# Autodesk Inventor assembly: owl1.1
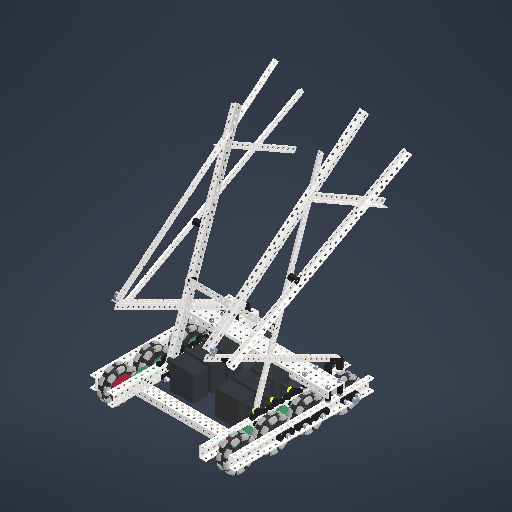
[picture p0: Inventor's stored thumbnail of the model, 512x512]
Saved by Autodesk Inventor 2026 (Build 300175000, 175)
## iProperties
Created: 2025-05-12
Part Number: owl1.1
Document SubType Name: Assembly
Designer: modni
Author: modni
## Documents named in this file (57)
- C:\Vex_cads\owl1.1.iam
- C:\Vex_cads\VEX-CAD-Inventor-1.4.2\Structure\C Channel\Aluminum 1x2x1\Alu C 1x2x1x24.ipt
- C:\Vex_cads\VEX-CAD-Inventor-1.4.2\Motion\Shaft LS\Bearing Flat.ipt
- C:\Vex_cads\VEX-CAD-Inventor-1.4.2\Structure\Hardware\Nut Thin Nylock.ipt
- C:\Vex_cads\VEX-CAD-Inventor-1.4.2\Structure\C Channel\Aluminum 1x3x1\Alu C 1x3x1x25.ipt
- C:\Vex_cads\VEX-CAD-Inventor-1.4.2\Structure\Hardware\Screw Steel - Star\SScrew Star Smooth 1.250.ipt
- C:\Vex_cads\VEX-CAD-Inventor-1.4.2\Structure\Hardware\Screw Steel - Star.ipt
- C:\Vex_cads\VEX-CAD-Inventor-1.4.2\Structure\Hardware\Nut Keps.ipt
- C:\Vex_cads\VEX-CAD-Inventor-1.4.2\Motion\Spacers\Spacer Nylon .375 OD\NSpacer .375 OD x .375.ipt
- C:\Vex_cads\VEX-CAD-Inventor-1.4.2\Motion\Spacers\Spacer Nylon .375 OD.ipt
- C:\Vex_cads\VEX-CAD-Inventor-1.4.2\Structure\C Channel\Aluminum 1x2x1\Alu C 1x2x1x25.ipt
- C:\Vex_cads\VEX-CAD-Inventor-1.4.2\Motion\Shaft LS\Shaft Collar Metal\Shaft Collar Set Screw.ipt
- C:\Vex_cads\VEX-CAD-Inventor-1.4.2\Motion\Spacers\Spacer Nylon .375 OD\NSpacer .375 OD x .250.ipt
- C:\Vex_cads\VEX-CAD-Inventor-1.4.2\Structure\Hardware\Nut Nylock.ipt
- C:\Vex_cads\VEX-CAD-Inventor-1.4.2\Motion\Shaft LS\LS Pillow Bearing Block.ipt
- C:\Vex_cads\VEX-CAD-Inventor-1.4.2\Electronics\V5 Simple Motor.ipt
- C:\Vex_cads\VEX-CAD-Inventor-1.4.2\Motion\Spacers\Washer Teflon\TWasher .375 OD x .04000.ipt
- C:\Vex_cads\VEX-CAD-Inventor-1.4.2\Motion\Spacers\Washer Teflon.ipt
- C:\Vex_cads\VEX-CAD-Inventor-1.4.2\Motion\Spacers\Washer Steel\SWasher .375 OD x .015625.ipt
- C:\Vex_cads\VEX-CAD-Inventor-1.4.2\Motion\Spacers\Washer Steel.ipt
- C:\Vex_cads\VEX-CAD-Inventor-1.4.2\Motion\Wheels\Omni Wheel\2.75 Omni AS, Circle.iam
- C:\Vex_cads\VEX-CAD-Inventor-1.4.2\Motion\Wheels\Omni Wheel.iam
- C:\Vex_cads\VEX-CAD-Inventor-1.4.2\Motion\Gears\HS Gear\HS 36T Gear, Circle.iam
- C:\Vex_cads\VEX-CAD-Inventor-1.4.2\Motion\Gears\HS Gear.iam
- C:\Vex_cads\VEX-CAD-Inventor-1.4.2\Structure\C Channel\Aluminum 1x2x1\Alu C 1x2x1x17.ipt
- C:\Vex_cads\VEX-CAD-Inventor-1.4.2\Motion\Spacers\Spacer Nylon .375 OD\NSpacer .375 OD x .500.ipt
- C:\Vex_cads\VEX-CAD-Inventor-1.4.2\Motion\Gears\LS 36T Gear.ipt
- C:\Vex_cads\VEX-CAD-Inventor-1.4.2\Motion\Wheels\Omni Wheel\2.75 Omni AS, Square.iam
- C:\Vex_cads\VEX-CAD-Inventor-1.4.2\Structure\C Channel\Aluminum 1x2x1\Alu C 1x2x1x24_MIR.ipt
- C:\Vex_cads\VEX-CAD-Inventor-1.4.2\Motion\Shaft LS\Bearing Flat_MIR.ipt
- C:\Vex_cads\VEX-CAD-Inventor-1.4.2\Structure\Hardware\Nut Thin Nylock_MIR.ipt
- C:\Vex_cads\VEX-CAD-Inventor-1.4.2\Structure\Hardware\Nut Keps_MIR.ipt
- C:\Vex_cads\VEX-CAD-Inventor-1.4.2\Structure\C Channel\Aluminum 1x2x1\Alu C 1x2x1x25_MIR.ipt
- C:\Vex_cads\VEX-CAD-Inventor-1.4.2\Motion\Shaft LS\Shaft Collar Metal\Shaft Collar Set Screw_MIR.ipt
- C:\Vex_cads\VEX-CAD-Inventor-1.4.2\Structure\Hardware\Nut Nylock_MIR.ipt
- C:\Vex_cads\VEX-CAD-Inventor-1.4.2\Motion\Shaft LS\LS Pillow Bearing Block_MIR.ipt
- C:\Vex_cads\VEX-CAD-Inventor-1.4.2\Electronics\V5 Simple Motor_MIR.ipt
- C:\Vex_cads\VEX-CAD-Inventor-1.4.2\Motion\Wheels\Omni Wheel\2.75 Omni AS, Circle_MIR.iam
- C:\Vex_cads\VEX-CAD-Inventor-1.4.2\Motion\Gears\HS Gear\HS 36T Gear, Circle_MIR.iam
- C:\Vex_cads\VEX-CAD-Inventor-1.4.2\Motion\Gears\LS 36T Gear_MIR.ipt
- C:\Vex_cads\VEX-CAD-Inventor-1.4.2\Motion\Wheels\Omni Wheel\2.75 Omni AS, Square_MIR.iam
- C:\Vex_cads\VEX-CAD-Inventor-1.4.2\Motion\Spacers\Spacer Nylon .500 OD\NSpacer Black .500 OD x .500.ipt
- C:\Vex_cads\VEX-CAD-Inventor-1.4.2\Motion\Spacers\Spacer Nylon .500 OD.ipt
- C:\Vex_cads\VEX-CAD-Inventor-1.4.2\Motion\Spacers\Spacer Nylon .500 OD\NSpacer Black .500 OD x .125.ipt
- C:\Vex_cads\VEX-CAD-Inventor-1.4.2\Structure\Angle\Aluminum 1x1\Alu Angle 1x1x25.ipt
- C:\Vex_cads\VEX-CAD-Inventor-1.4.2\Structure\Angle\Aluminum 1x1\Alu Angle 1x1x35.ipt
- C:\Vex_cads\VEX-CAD-Inventor-1.4.2\Motion\Spacers\Spacer Nylon .375 OD\NSpacer .375 OD x .125.ipt
- C:\Vex_cads\VEX-CAD-Inventor-1.4.2\Motion\Spacers\Spacer Nylon .500 OD\NSpacer Black .500 OD x .375.ipt
- C:\Vex_cads\VEX-CAD-Inventor-1.4.2\Motion\Spacers\Spacer Nylon .500 OD\NSpacer Black .500 OD x .250.ipt
- C:\Vex_cads\VEX-CAD-Inventor-1.4.2\Motion\Shaft LS\Shaft Collar Metal\Shaft Collar No Screw.ipt
- C:\Vex_cads\VEX-CAD-Inventor-1.4.2\Structure\Angle\Aluminum 1x1\Alu Angle 1x1x15.ipt
- C:\Vex_cads\VEX-CAD-Inventor-1.4.2\Motion\Shaft LS\LS Pillow Bearing Block_MIR1.ipt
- C:\Vex_cads\VEX-CAD-Inventor-1.4.2\Structure\Angle\Aluminum 1x1\Alu Angle 1x1x25_MIR.ipt
- C:\Vex_cads\VEX-CAD-Inventor-1.4.2\Structure\Angle\Aluminum 1x1\Alu Angle 1x1x35_MIR.ipt
- C:\Vex_cads\VEX-CAD-Inventor-1.4.2\Motion\Shaft LS\Shaft Collar Metal\Shaft Collar No Screw_MIR.ipt
- C:\Vex_cads\VEX-CAD-Inventor-1.4.2\Structure\Hardware\Nut Keps_MIR1.ipt
- C:\Vex_cads\VEX-CAD-Inventor-1.4.2\Structure\Angle\Aluminum 1x1\Alu Angle 1x1x15_MIR.ipt
## Components (193 placed, 49 different names)
1. Alu C 1x2x1x24:1 — Mate:1, Mate:2, Mate:3, Mate:4, Insert:2, Insert:3, Insert:4, Insert:5, Symmetry:1
2. Bearing Flat:1 — Mate:1, Mate:6
3. Bearing Flat:2 — Mate:2, Mate:5
4. Bearing Flat:3 — Mate:3, Mate:7
5. Bearing Flat:4 — Mate:4, Mate:8, Insert:1, Insert:25
6. Nut Thin Nylock:1 — Mate:6
7. Nut Thin Nylock:2 — Mate:5
8. Nut Thin Nylock:3 — Mate:7
9. Nut Thin Nylock:4 — Insert:1
10. Nut Thin Nylock:5 — Mate:8
11. Alu C 1x3x1x25:1 — Insert:10, Insert:15, Insert:16, Insert:33, Insert:34, Insert:35, Insert:36
12. SScrew Star Smooth 1.250:1 — Insert:3
13. SScrew Star Smooth 1.250:2 — Insert:2
14. Nut Keps:1 — Insert:5, Insert:8
15. Nut Keps:2 — Insert:4, Insert:6
16. NSpacer .375 OD x .375:1 — Insert:6, Insert:7
17. NSpacer .375 OD x .375:2 — Insert:7
18. NSpacer .375 OD x .375:3 — Insert:9, Insert:10
19. NSpacer .375 OD x .375:4 — Insert:8, Insert:9
20. Alu C 1x2x1x25:1 — Insert:17, Insert:18, Insert:19, Insert:20, Insert:21, Insert:22, Insert:23, Insert:37, Insert:38, Insert:39, Insert:40, Insert:41, Insert:42, Insert:50, Insert:55, Insert:56, Insert:70, Insert:71, Insert:72, Insert:76, Insert:77, Insert:141, Insert:143
21. SScrew Star Smooth 1.250:3 — Insert:19
22. SScrew Star Smooth 1.250:4 — Insert:18
23. Nut Keps:3 — Insert:17
24. Nut Keps:4
25. NSpacer .375 OD x .375:5
26. NSpacer .375 OD x .375:6 — Insert:15
27. NSpacer .375 OD x .375:7 — Insert:16
28. NSpacer .375 OD x .375:8
29. Bearing Flat:5 — Insert:23, Insert:24
30. Bearing Flat:6 — Insert:22, Insert:31, Insert:32
31. Bearing Flat:7 — Insert:21, Insert:29, Insert:30
32. Bearing Flat:8 — Insert:20, Insert:27, Insert:28
33. Shaft Collar Set Screw:1 — Insert:24
34. Shaft Collar Set Screw:2 — Insert:26
35. NSpacer .375 OD x .250:9 — Insert:25, Insert:26
36. Nut Nylock:1 — Insert:32
37. Nut Nylock:2 — Insert:31
38. Nut Nylock:3 — Insert:30
39. Nut Nylock:4 — Insert:29
40. Nut Nylock:5 — Insert:27
41. Nut Nylock:6 — Insert:28
42. Nut Thin Nylock:6 — Insert:33
43. Nut Thin Nylock:7 — Insert:34
44. Nut Thin Nylock:8 — Insert:35
45. Nut Thin Nylock:9 — Insert:36
46. LS Pillow Bearing Block:1 — Insert:37, Insert:147
47. LS Pillow Bearing Block:2 — Insert:38
48. LS Pillow Bearing Block:3 — Insert:39
49. V5 Simple Motor:1 — Insert:40
50. V5 Simple Motor:2 — Insert:41
51. V5 Simple Motor:3 — Insert:42
52. NSpacer .375 OD x .250:10 — Insert:49
53. TWasher .375 OD x .04000:1 — Insert:43, Insert:54
54. SWasher .375 OD x .015625:1 — Insert:43, Insert:51
55. 2.75 Omni AS, Circle:1 [sub-assembly] — Insert:49, Insert:52
56. Nut Keps:5 — Insert:50, Insert:53
57. HS 36T Gear, Circle:1 [sub-assembly] — Insert:51, Insert:52
58. NSpacer .375 OD x .375:11 — Insert:53, Insert:54
59. Alu C 1x2x1x17:1 — Insert:55
60. NSpacer .375 OD x .250:14 — Insert:60, Insert:61
61. NSpacer .375 OD x .500:12 — Insert:56, Insert:57
62. LS 36T Gear:1 — Insert:57, Insert:60
63. 2.75 Omni AS, Square:3 [sub-assembly] — Insert:59, Insert:61
64. NSpacer .375 OD x .375:13 — Insert:59
65. NSpacer .375 OD x .500:15 — Insert:70
66. LS 36T Gear:2
67. 2.75 Omni AS, Square:4 [sub-assembly]
68. NSpacer .375 OD x .375:16
69. NSpacer .375 OD x .250:17
70. NSpacer .375 OD x .500:18 — Insert:71
71. LS 36T Gear:3
72. 2.75 Omni AS, Square:5 [sub-assembly]
73. NSpacer .375 OD x .375:19
74. NSpacer .375 OD x .250:20
75. NSpacer .375 OD x .500:21 — Insert:72, Insert:73
76. LS 36T Gear:4 — Insert:73
77. NSpacer .375 OD x .500:22 — Insert:77
78. LS 36T Gear:5
79. NSpacer .375 OD x .500:23 — Insert:76
80. LS 36T Gear:6
81. Alu C 1x2x1x24_MIR:1 — Mate:9, Mate:10, Mate:11, Mate:12, Insert:79, Insert:80, Insert:81, Insert:82, Symmetry:1
82. Bearing Flat_MIR:1 — Mate:9, Mate:13
83. Bearing Flat_MIR:2 — Mate:10, Mate:14
84. Bearing Flat_MIR:3 — Mate:11, Mate:15
85. Bearing Flat_MIR:4 — Mate:12, Insert:78, Mate:16, Insert:100
86. Nut Thin Nylock_MIR:1 — Mate:13
87. Nut Thin Nylock_MIR:2 — Mate:14
88. Nut Thin Nylock_MIR:3 — Mate:15
89. Nut Thin Nylock_MIR:4 — Insert:78
90. Nut Thin Nylock_MIR:5 — Mate:16
91. SScrew Star Smooth 1.250:5 — Insert:79
92. SScrew Star Smooth 1.250:6 — Insert:80
93. Nut Keps_MIR:1 — Insert:81, Insert:86
94. Nut Keps_MIR:2 — Insert:82, Insert:83
95. NSpacer .375 OD x .375:24 — Insert:83, Insert:84
96. NSpacer .375 OD x .375:25 — Insert:84
97. NSpacer .375 OD x .375:26 — Insert:85
98. NSpacer .375 OD x .375:27 — Insert:85, Insert:86
99. Alu C 1x2x1x25_MIR:1 — Insert:87, Insert:88, Insert:89, Insert:94, Insert:95, Insert:96, Insert:97, Insert:107, Insert:108, Insert:109, Insert:110, Insert:111, Insert:112, Insert:115, Insert:120, Insert:125, Insert:130, Insert:135, Insert:137, Insert:139
100. SScrew Star Smooth 1.250:7 — Insert:87
101. SScrew Star Smooth 1.250:8 — Insert:88
102. Nut Keps_MIR:3 — Insert:89, Insert:93
103. Nut Keps_MIR:4 — Insert:90
104. NSpacer .375 OD x .375:28 — Insert:90, Insert:91
105. NSpacer .375 OD x .375:29 — Insert:91
106. NSpacer .375 OD x .375:30 — Insert:92
107. NSpacer .375 OD x .375:31 — Insert:92, Insert:93
108. Bearing Flat_MIR:5 — Insert:94, Insert:98
109. Bearing Flat_MIR:6 — Insert:95, Insert:101, Insert:102
110. Bearing Flat_MIR:7 — Insert:96, Insert:103, Insert:104
111. Bearing Flat_MIR:8 — Insert:97, Insert:105, Insert:106
112. Shaft Collar Set Screw_MIR:1 — Insert:98
113. Shaft Collar Set Screw_MIR:2 — Insert:99
114. NSpacer .375 OD x .250:32 — Insert:99, Insert:100
115. Nut Nylock_MIR:1 — Insert:101
116. Nut Nylock_MIR:2 — Insert:102
117. Nut Nylock_MIR:3 — Insert:103
118. Nut Nylock_MIR:4 — Insert:104
119. Nut Nylock_MIR:5 — Insert:105
120. Nut Nylock_MIR:6 — Insert:106
121. Nut Thin Nylock_MIR:6
122. Nut Thin Nylock_MIR:7
123. Nut Thin Nylock_MIR:8
124. Nut Thin Nylock_MIR:9
125. LS Pillow Bearing Block_MIR:1 — Insert:107
126. LS Pillow Bearing Block_MIR:2 — Insert:108
127. LS Pillow Bearing Block_MIR:3 — Insert:109
128. V5 Simple Motor_MIR:1 — Insert:110
129. V5 Simple Motor_MIR:2 — Insert:111
130. V5 Simple Motor_MIR:3 — Insert:112
131. NSpacer .375 OD x .250:33 — Insert:114
132. TWasher .375 OD x .04000:2 — Insert:113, Insert:118
133. SWasher .375 OD x .015625:2 — Insert:113, Insert:117
134. 2.75 Omni AS, Circle_MIR:1 [sub-assembly] — Insert:114, Insert:116
135. Nut Keps_MIR:5 — Insert:115, Insert:119
136. HS 36T Gear, Circle_MIR:1 [sub-assembly] — Insert:116, Insert:117
137. NSpacer .375 OD x .375:34 — Insert:118, Insert:119
138. NSpacer .375 OD x .250:35 — Insert:123, Insert:124
139. NSpacer .375 OD x .500:36 — Insert:120, Insert:121
140. LS 36T Gear_MIR:1 — Insert:121, Insert:124
141. 2.75 Omni AS, Square_MIR:1 [sub-assembly] — Insert:122, Insert:123
142. NSpacer .375 OD x .375:37 — Insert:122
143. NSpacer .375 OD x .500:38 — Insert:125, Insert:126
144. LS 36T Gear_MIR:2 — Insert:126, Insert:129
145. 2.75 Omni AS, Square_MIR:2 [sub-assembly] — Insert:127, Insert:128
146. NSpacer .375 OD x .375:39 — Insert:127
147. NSpacer .375 OD x .250:40 — Insert:128, Insert:129
148. NSpacer .375 OD x .500:41 — Insert:130, Insert:131
149. LS 36T Gear_MIR:3 — Insert:131, Insert:134
150. 2.75 Omni AS, Square_MIR:3 [sub-assembly] — Insert:132, Insert:133
151. NSpacer .375 OD x .375:42 — Insert:132
152. NSpacer .375 OD x .250:43 — Insert:133, Insert:134
153. NSpacer .375 OD x .500:44 — Insert:135, Insert:136
154. LS 36T Gear_MIR:4 — Insert:136
155. NSpacer .375 OD x .500:45 — Insert:137, Insert:138
156. LS 36T Gear_MIR:5 — Insert:138
157. NSpacer .375 OD x .500:46 — Insert:139, Insert:140
158. LS 36T Gear_MIR:6 — Insert:140
159. NSpacer Black .500 OD x .500:1 — Insert:141, Insert:142
160. NSpacer Black .500 OD x .500:2 — Insert:143, Insert:144
161. NSpacer Black .500 OD x .125:3 — Insert:142, Insert:145
162. NSpacer Black .500 OD x .125:4 — Insert:144
163. LS Pillow Bearing Block:4 — Insert:145, Insert:146
164. Alu Angle 1x1x25:1 — Insert:146, Insert:149, Insert:150, Insert:154
165. Alu Angle 1x1x35:1 — Insert:148, Insert:149, Insert:152, Insert:157, Insert:172
166. NSpacer .375 OD x .125:47 — Insert:147, Insert:148
167. Alu Angle 1x1x35:2 — Insert:151
168. NSpacer .375 OD x .500:48 — Insert:150, Insert:151
169. NSpacer Black .500 OD x .375:6 — Insert:153
170. NSpacer Black .500 OD x .250:7 — Insert:152, Insert:153
171. Alu Angle 1x1x35:3 — Insert:156
172. Shaft Collar No Screw:1 — Insert:155, Insert:156
173. Nut Keps:6 — Insert:154, Insert:155
174. Alu Angle 1x1x15:1 — Insert:157
175. NSpacer Black .500 OD x .500:8 — Insert:158
176. NSpacer Black .500 OD x .500:9 — Insert:159
177. NSpacer Black .500 OD x .125:10 — Insert:158, Insert:160
178. NSpacer Black .500 OD x .125:11 — Insert:159
179. LS Pillow Bearing Block_MIR1:1 — Insert:160, Insert:161
180. Alu Angle 1x1x25_MIR:1 — Insert:161, Insert:162, Insert:165, Insert:170
181. Alu Angle 1x1x35_MIR:1 — Insert:162, Insert:163, Insert:167, Insert:171, Insert:173
182. NSpacer .375 OD x .125:49 — Insert:163
183. Alu Angle 1x1x35_MIR:2 — Insert:164
184. NSpacer .375 OD x .500:50 — Insert:164, Insert:165
185. NSpacer Black .500 OD x .375:12 — Insert:166
186. NSpacer Black .500 OD x .250:13 — Insert:166, Insert:167
187. Alu Angle 1x1x35_MIR:3 — Insert:168
188. Shaft Collar No Screw_MIR:1 — Insert:168, Insert:169
189. Nut Keps_MIR1:1 — Insert:169, Insert:170
190. Alu Angle 1x1x15_MIR:1 — Insert:171
191. NSpacer .375 OD x .500:51 — Insert:172, Insert:174
192. NSpacer .375 OD x .500:52 — Insert:173, Insert:175
193. Alu Angle 1x1x15:2 — Insert:174, Insert:175
## Relationships (186: Insert 169, Mate 16, Symmetry 1)
- Mate:1: Alu C 1x2x1x24:1 ↔ Bearing Flat:1
- Mate:2: Alu C 1x2x1x24:1 ↔ Bearing Flat:2
- Mate:3: Alu C 1x2x1x24:1 ↔ Bearing Flat:3
- Mate:4: Alu C 1x2x1x24:1 ↔ Bearing Flat:4
- Mate:5: Bearing Flat:2 ↔ Nut Thin Nylock:2
- Mate:6: Bearing Flat:1 ↔ Nut Thin Nylock:1
- Mate:7: Bearing Flat:3 ↔ Nut Thin Nylock:3
- Mate:8: Bearing Flat:4 ↔ Nut Thin Nylock:5
- Insert:1: Bearing Flat:4 ↔ Nut Thin Nylock:4
- Insert:2: Alu C 1x2x1x24:1 ↔ SScrew Star Smooth 1.250:2
- Insert:3: Alu C 1x2x1x24:1 ↔ SScrew Star Smooth 1.250:1
- Insert:4: Alu C 1x2x1x24:1 ↔ Nut Keps:2
- Insert:5: Alu C 1x2x1x24:1 ↔ Nut Keps:1
- Insert:6: Nut Keps:2 ↔ NSpacer .375 OD x .375:1
- Insert:7: NSpacer .375 OD x .375:1 ↔ NSpacer .375 OD x .375:2
- Insert:8: Nut Keps:1 ↔ NSpacer .375 OD x .375:4
- Insert:9: NSpacer .375 OD x .375:3 ↔ NSpacer .375 OD x .375:4
- Insert:10: Alu C 1x3x1x25:1 ↔ NSpacer .375 OD x .375:3
- [Insert]: Nut Keps:4 ↔ NSpacer .375 OD x .375:5
- [Insert]: NSpacer .375 OD x .375:5 ↔ NSpacer .375 OD x .375:6
- [Insert]: Nut Keps:3 ↔ NSpacer .375 OD x .375:8
- [Insert]: NSpacer .375 OD x .375:7 ↔ NSpacer .375 OD x .375:8
- Insert:15: Alu C 1x3x1x25:1 ↔ NSpacer .375 OD x .375:6
- Insert:16: Alu C 1x3x1x25:1 ↔ NSpacer .375 OD x .375:7
- Insert:17: Alu C 1x2x1x25:1 ↔ Nut Keps:3
- Insert:18: Alu C 1x2x1x25:1 ↔ SScrew Star Smooth 1.250:4
- Insert:19: Alu C 1x2x1x25:1 ↔ SScrew Star Smooth 1.250:3
- Insert:20: Alu C 1x2x1x25:1 ↔ Bearing Flat:8
- Insert:21: Alu C 1x2x1x25:1 ↔ Bearing Flat:7
- Insert:22: Alu C 1x2x1x25:1 ↔ Bearing Flat:6
- Insert:23: Alu C 1x2x1x25:1 ↔ Bearing Flat:5
- Insert:24: Bearing Flat:5 ↔ Shaft Collar Set Screw:1
- Insert:25: Bearing Flat:4 ↔ NSpacer .375 OD x .250:9
- Insert:26: Shaft Collar Set Screw:2 ↔ NSpacer .375 OD x .250:9
- Insert:27: Bearing Flat:8 ↔ Nut Nylock:5
- Insert:28: Bearing Flat:8 ↔ Nut Nylock:6
- Insert:29: Bearing Flat:7 ↔ Nut Nylock:4
- Insert:30: Bearing Flat:7 ↔ Nut Nylock:3
- Insert:31: Bearing Flat:6 ↔ Nut Nylock:2
- Insert:32: Bearing Flat:6 ↔ Nut Nylock:1
- Insert:33: Alu C 1x3x1x25:1 ↔ Nut Thin Nylock:6
- Insert:34: Alu C 1x3x1x25:1 ↔ Nut Thin Nylock:7
- Insert:35: Alu C 1x3x1x25:1 ↔ Nut Thin Nylock:8
- Insert:36: Alu C 1x3x1x25:1 ↔ Nut Thin Nylock:9
- Insert:37: Alu C 1x2x1x25:1 ↔ LS Pillow Bearing Block:1
- Insert:38: Alu C 1x2x1x25:1 ↔ LS Pillow Bearing Block:2
- Insert:39: Alu C 1x2x1x25:1 ↔ LS Pillow Bearing Block:3
- Insert:40: Alu C 1x2x1x25:1 ↔ V5 Simple Motor:1
- Insert:41: Alu C 1x2x1x25:1 ↔ V5 Simple Motor:2
- Insert:42: Alu C 1x2x1x25:1 ↔ V5 Simple Motor:3
- Insert:43: TWasher .375 OD x .04000:1 ↔ SWasher .375 OD x .015625:1
- Insert:49: NSpacer .375 OD x .250:10 ↔ 2.75 Omni AS, Circle:1
- Insert:50: Alu C 1x2x1x25:1 ↔ Nut Keps:5
- Insert:51: SWasher .375 OD x .015625:1 ↔ HS 36T Gear, Circle:1
- Insert:52: 2.75 Omni AS, Circle:1 ↔ HS 36T Gear, Circle:1
- Insert:53: Nut Keps:5 ↔ NSpacer .375 OD x .375:11
- Insert:54: TWasher .375 OD x .04000:1 ↔ NSpacer .375 OD x .375:11
- Insert:55: Alu C 1x2x1x25:1 ↔ Alu C 1x2x1x17:1
- Insert:56: Alu C 1x2x1x25:1 ↔ NSpacer .375 OD x .500:12
- Insert:57: NSpacer .375 OD x .500:12 ↔ LS 36T Gear:1
- Insert:59: 2.75 Omni AS, Square:3 ↔ NSpacer .375 OD x .375:13
- Insert:60: NSpacer .375 OD x .250:14 ↔ LS 36T Gear:1
- Insert:61: NSpacer .375 OD x .250:14 ↔ 2.75 Omni AS, Square:3
- [Insert]: NSpacer .375 OD x .500:15 ↔ LS 36T Gear:2
- [Insert]: 2.75 Omni AS, Square:4 ↔ NSpacer .375 OD x .375:16
- [Insert]: LS 36T Gear:2 ↔ NSpacer .375 OD x .250:17
- [Insert]: 2.75 Omni AS, Square:4 ↔ NSpacer .375 OD x .250:17
- [Insert]: NSpacer .375 OD x .500:18 ↔ LS 36T Gear:3
- [Insert]: 2.75 Omni AS, Square:5 ↔ NSpacer .375 OD x .375:19
- [Insert]: LS 36T Gear:3 ↔ NSpacer .375 OD x .250:20
- [Insert]: 2.75 Omni AS, Square:5 ↔ NSpacer .375 OD x .250:20
- Insert:70: Alu C 1x2x1x25:1 ↔ NSpacer .375 OD x .500:15
- Insert:71: Alu C 1x2x1x25:1 ↔ NSpacer .375 OD x .500:18
- Insert:72: Alu C 1x2x1x25:1 ↔ NSpacer .375 OD x .500:21
- Insert:73: NSpacer .375 OD x .500:21 ↔ LS 36T Gear:4
- [Insert]: NSpacer .375 OD x .500:22 ↔ LS 36T Gear:5
- [Insert]: NSpacer .375 OD x .500:23 ↔ LS 36T Gear:6
- Insert:76: Alu C 1x2x1x25:1 ↔ NSpacer .375 OD x .500:23
- Insert:77: Alu C 1x2x1x25:1 ↔ NSpacer .375 OD x .500:22
- Mate:9: Alu C 1x2x1x24_MIR:1 ↔ Bearing Flat_MIR:1
- Mate:10: Alu C 1x2x1x24_MIR:1 ↔ Bearing Flat_MIR:2
- Mate:11: Alu C 1x2x1x24_MIR:1 ↔ Bearing Flat_MIR:3
- Mate:12: Alu C 1x2x1x24_MIR:1 ↔ Bearing Flat_MIR:4
- Mate:13: Bearing Flat_MIR:1 ↔ Nut Thin Nylock_MIR:1
- Mate:14: Bearing Flat_MIR:2 ↔ Nut Thin Nylock_MIR:2
- Mate:15: Bearing Flat_MIR:3 ↔ Nut Thin Nylock_MIR:3
- Insert:78: Bearing Flat_MIR:4 ↔ Nut Thin Nylock_MIR:4
- Mate:16: Bearing Flat_MIR:4 ↔ Nut Thin Nylock_MIR:5
- Insert:79: Alu C 1x2x1x24_MIR:1 ↔ SScrew Star Smooth 1.250:5
- Insert:80: Alu C 1x2x1x24_MIR:1 ↔ SScrew Star Smooth 1.250:6
- Insert:81: Alu C 1x2x1x24_MIR:1 ↔ Nut Keps_MIR:1
- Insert:82: Alu C 1x2x1x24_MIR:1 ↔ Nut Keps_MIR:2
- Insert:83: Nut Keps_MIR:2 ↔ NSpacer .375 OD x .375:24
- Insert:84: NSpacer .375 OD x .375:24 ↔ NSpacer .375 OD x .375:25
- Insert:85: NSpacer .375 OD x .375:26 ↔ NSpacer .375 OD x .375:27
- Insert:86: Nut Keps_MIR:1 ↔ NSpacer .375 OD x .375:27
- Insert:87: Alu C 1x2x1x25_MIR:1 ↔ SScrew Star Smooth 1.250:7
- Insert:88: Alu C 1x2x1x25_MIR:1 ↔ SScrew Star Smooth 1.250:8
- Insert:89: Alu C 1x2x1x25_MIR:1 ↔ Nut Keps_MIR:3
- Insert:90: Nut Keps_MIR:4 ↔ NSpacer .375 OD x .375:28
- Insert:91: NSpacer .375 OD x .375:28 ↔ NSpacer .375 OD x .375:29
- Insert:92: NSpacer .375 OD x .375:30 ↔ NSpacer .375 OD x .375:31
- Insert:93: Nut Keps_MIR:3 ↔ NSpacer .375 OD x .375:31
- Insert:94: Alu C 1x2x1x25_MIR:1 ↔ Bearing Flat_MIR:5
- Insert:95: Alu C 1x2x1x25_MIR:1 ↔ Bearing Flat_MIR:6
- Insert:96: Alu C 1x2x1x25_MIR:1 ↔ Bearing Flat_MIR:7
- Insert:97: Alu C 1x2x1x25_MIR:1 ↔ Bearing Flat_MIR:8
- Insert:98: Bearing Flat_MIR:5 ↔ Shaft Collar Set Screw_MIR:1
- Insert:99: Shaft Collar Set Screw_MIR:2 ↔ NSpacer .375 OD x .250:32
- Insert:100: Bearing Flat_MIR:4 ↔ NSpacer .375 OD x .250:32
- Insert:101: Bearing Flat_MIR:6 ↔ Nut Nylock_MIR:1
- Insert:102: Bearing Flat_MIR:6 ↔ Nut Nylock_MIR:2
- Insert:103: Bearing Flat_MIR:7 ↔ Nut Nylock_MIR:3
- Insert:104: Bearing Flat_MIR:7 ↔ Nut Nylock_MIR:4
- Insert:105: Bearing Flat_MIR:8 ↔ Nut Nylock_MIR:5
- Insert:106: Bearing Flat_MIR:8 ↔ Nut Nylock_MIR:6
- Insert:107: Alu C 1x2x1x25_MIR:1 ↔ LS Pillow Bearing Block_MIR:1
- Insert:108: Alu C 1x2x1x25_MIR:1 ↔ LS Pillow Bearing Block_MIR:2
- Insert:109: Alu C 1x2x1x25_MIR:1 ↔ LS Pillow Bearing Block_MIR:3
- Insert:110: Alu C 1x2x1x25_MIR:1 ↔ V5 Simple Motor_MIR:1
- Insert:111: Alu C 1x2x1x25_MIR:1 ↔ V5 Simple Motor_MIR:2
- Insert:112: Alu C 1x2x1x25_MIR:1 ↔ V5 Simple Motor_MIR:3
- Insert:113: TWasher .375 OD x .04000:2 ↔ SWasher .375 OD x .015625:2
- Insert:114: NSpacer .375 OD x .250:33 ↔ 2.75 Omni AS, Circle_MIR:1
- Insert:115: Alu C 1x2x1x25_MIR:1 ↔ Nut Keps_MIR:5
- Insert:116: 2.75 Omni AS, Circle_MIR:1 ↔ HS 36T Gear, Circle_MIR:1
- Insert:117: SWasher .375 OD x .015625:2 ↔ HS 36T Gear, Circle_MIR:1
- Insert:118: TWasher .375 OD x .04000:2 ↔ NSpacer .375 OD x .375:34
- Insert:119: Nut Keps_MIR:5 ↔ NSpacer .375 OD x .375:34
- Insert:120: Alu C 1x2x1x25_MIR:1 ↔ NSpacer .375 OD x .500:36
- Insert:121: NSpacer .375 OD x .500:36 ↔ LS 36T Gear_MIR:1
- Insert:122: 2.75 Omni AS, Square_MIR:1 ↔ NSpacer .375 OD x .375:37
- Insert:123: NSpacer .375 OD x .250:35 ↔ 2.75 Omni AS, Square_MIR:1
- Insert:124: NSpacer .375 OD x .250:35 ↔ LS 36T Gear_MIR:1
- Insert:125: Alu C 1x2x1x25_MIR:1 ↔ NSpacer .375 OD x .500:38
- Insert:126: NSpacer .375 OD x .500:38 ↔ LS 36T Gear_MIR:2
- Insert:127: 2.75 Omni AS, Square_MIR:2 ↔ NSpacer .375 OD x .375:39
- Insert:128: 2.75 Omni AS, Square_MIR:2 ↔ NSpacer .375 OD x .250:40
- Insert:129: LS 36T Gear_MIR:2 ↔ NSpacer .375 OD x .250:40
- Insert:130: Alu C 1x2x1x25_MIR:1 ↔ NSpacer .375 OD x .500:41
- Insert:131: NSpacer .375 OD x .500:41 ↔ LS 36T Gear_MIR:3
- Insert:132: 2.75 Omni AS, Square_MIR:3 ↔ NSpacer .375 OD x .375:42
- Insert:133: 2.75 Omni AS, Square_MIR:3 ↔ NSpacer .375 OD x .250:43
- Insert:134: LS 36T Gear_MIR:3 ↔ NSpacer .375 OD x .250:43
- Insert:135: Alu C 1x2x1x25_MIR:1 ↔ NSpacer .375 OD x .500:44
- Insert:136: NSpacer .375 OD x .500:44 ↔ LS 36T Gear_MIR:4
- Insert:137: Alu C 1x2x1x25_MIR:1 ↔ NSpacer .375 OD x .500:45
- Insert:138: NSpacer .375 OD x .500:45 ↔ LS 36T Gear_MIR:5
- Insert:139: Alu C 1x2x1x25_MIR:1 ↔ NSpacer .375 OD x .500:46
- Insert:140: NSpacer .375 OD x .500:46 ↔ LS 36T Gear_MIR:6
- Insert:141: Alu C 1x2x1x25:1 ↔ NSpacer Black .500 OD x .500:1
- Insert:142: NSpacer Black .500 OD x .500:1 ↔ NSpacer Black .500 OD x .125:3
- Insert:143: Alu C 1x2x1x25:1 ↔ NSpacer Black .500 OD x .500:2
- Insert:144: NSpacer Black .500 OD x .500:2 ↔ NSpacer Black .500 OD x .125:4
- Insert:145: NSpacer Black .500 OD x .125:3 ↔ LS Pillow Bearing Block:4
- Insert:146: LS Pillow Bearing Block:4 ↔ Alu Angle 1x1x25:1
- Insert:147: LS Pillow Bearing Block:1 ↔ NSpacer .375 OD x .125:47
- Insert:148: Alu Angle 1x1x35:1 ↔ NSpacer .375 OD x .125:47
- Insert:149: Alu Angle 1x1x25:1 ↔ Alu Angle 1x1x35:1
- Insert:150: Alu Angle 1x1x25:1 ↔ NSpacer .375 OD x .500:48
- Insert:151: Alu Angle 1x1x35:2 ↔ NSpacer .375 OD x .500:48
- Insert:152: Alu Angle 1x1x35:1 ↔ NSpacer Black .500 OD x .250:7
- Insert:153: NSpacer Black .500 OD x .375:6 ↔ NSpacer Black .500 OD x .250:7
- Insert:154: Alu Angle 1x1x25:1 ↔ Nut Keps:6
- Insert:155: Shaft Collar No Screw:1 ↔ Nut Keps:6
- Insert:156: Alu Angle 1x1x35:3 ↔ Shaft Collar No Screw:1
- Insert:157: Alu Angle 1x1x35:1 ↔ Alu Angle 1x1x15:1
- Symmetry:1: Alu C 1x2x1x24:1 ↔ Alu C 1x2x1x24_MIR:1
- Insert:158: NSpacer Black .500 OD x .500:8 ↔ NSpacer Black .500 OD x .125:10
- Insert:159: NSpacer Black .500 OD x .500:9 ↔ NSpacer Black .500 OD x .125:11
- Insert:160: NSpacer Black .500 OD x .125:10 ↔ LS Pillow Bearing Block_MIR1:1
- Insert:161: LS Pillow Bearing Block_MIR1:1 ↔ Alu Angle 1x1x25_MIR:1
- Insert:162: Alu Angle 1x1x25_MIR:1 ↔ Alu Angle 1x1x35_MIR:1
- Insert:163: Alu Angle 1x1x35_MIR:1 ↔ NSpacer .375 OD x .125:49
- Insert:164: Alu Angle 1x1x35_MIR:2 ↔ NSpacer .375 OD x .500:50
- Insert:165: Alu Angle 1x1x25_MIR:1 ↔ NSpacer .375 OD x .500:50
- Insert:166: NSpacer Black .500 OD x .375:12 ↔ NSpacer Black .500 OD x .250:13
- Insert:167: Alu Angle 1x1x35_MIR:1 ↔ NSpacer Black .500 OD x .250:13
- Insert:168: Alu Angle 1x1x35_MIR:3 ↔ Shaft Collar No Screw_MIR:1
- Insert:169: Shaft Collar No Screw_MIR:1 ↔ Nut Keps_MIR1:1
- Insert:170: Alu Angle 1x1x25_MIR:1 ↔ Nut Keps_MIR1:1
- Insert:171: Alu Angle 1x1x35_MIR:1 ↔ Alu Angle 1x1x15_MIR:1
- Insert:172: Alu Angle 1x1x35:1 ↔ NSpacer .375 OD x .500:51
- Insert:173: Alu Angle 1x1x35_MIR:1 ↔ NSpacer .375 OD x .500:52
- Insert:174: NSpacer .375 OD x .500:51 ↔ Alu Angle 1x1x15:2
- Insert:175: NSpacer .375 OD x .500:52 ↔ Alu Angle 1x1x15:2
## Named parameters: d18_d13 = 0 mm, d19_d14 = 0 mm, d20_d15 = 0 mm, d21_d16 = 0 mm, d79_d77 = 0 mm, d80_d78 = 0 mm, d81_d65 = 0 mm, d82_d67 = 0 mm, d83_d77 = 0 mm, d84_d78 = 0 mm, d85_d65 = 0 mm, d86_d67 = 0 mm, d91_d90 = 0 mm, d92_d90 = 0 mm
